# Autodesk Inventor assembly: rig
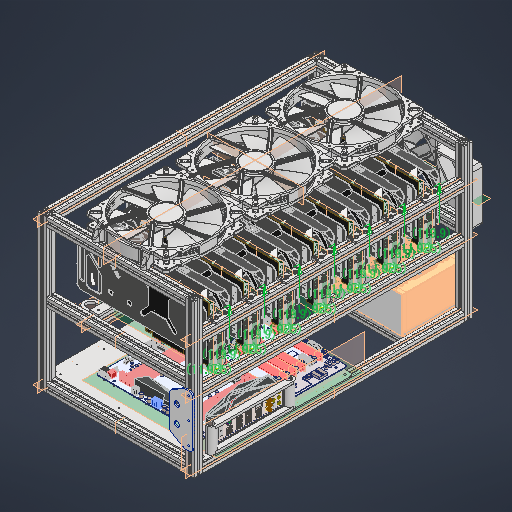
[picture p0: Inventor's stored thumbnail of the model, 512x512]
Saved by Autodesk Inventor 2026.2 (Build 302298010, 298A)
## iProperties
Created: 2026-05-30
Part Number: rig
Document SubType Name: Assembly
Designer: nyxeon
Author: nyxeon
## Documents named in this file (16)
- C:\Users\nyxeon\Documents\CAD\Inventor\eatx_case\robocup\rig.iam
- C:\Users\nyxeon\Documents\CAD\Inventor\eatx_case\robocup\l600.ipt
- C:\Users\nyxeon\Documents\CAD\Inventor\eatx_case\robocup\l320.ipt
- C:\Users\nyxeon\Documents\CAD\Inventor\eatx_case\robocup\l350.ipt
- C:\Users\nyxeon\Documents\CAD\Inventor\eatx_case\robocup\fan_unit_02.iam
- C:\Users\nyxeon\Documents\CAD\Inventor\eatx_case\robocup\fan_unit_01.iam
- C:\Users\nyxeon\Documents\CAD\Inventor\eatx_case\robocup\layout.iam
- C:\Users\nyxeon\Documents\CAD\Inventor\eatx_case\robocup\power_sync_module_case.ipt
- C:\Users\nyxeon\Documents\CAD\Inventor\eatx_case\robocup\power_sync_module_case_02.ipt
- C:\Users\nyxeon\Documents\CAD\Inventor\eatx_case\robocup\gpu_hold_plate.ipt
- C:\Users\nyxeon\Documents\CAD\Inventor\eatx_case\robocup\gpu_cable_holder.ipt
- C:\Users\nyxeon\Documents\CAD\Inventor\eatx_case\eatx_slim\resources\gpu\ASUS TUF RTX 3070 ti.iam
- C:\Users\nyxeon\Documents\CAD\Inventor\eatx_case\eatx_slim\resources\powersupply\ATX Power Supply v1.0.iam
- C:\Users\nyxeon\Documents\CAD\Inventor\eatx_case\robocup\gpu_support.ipt
- C:\Users\nyxeon\Documents\CAD\Inventor\eatx_case\robocup\atx_power_holder.ipt
- C:\Users\nyxeon\Documents\CAD\Inventor\eatx_case\robocup\robocup_power_sw_plate.ipt
## Components (49 placed, 15 different names)
1. l600:1 — フラッシュ:1, メイト:1, フラッシュ:2, メイト:2, フラッシュ:3, フラッシュ:4, メイト:43, フラッシュ:40
2. l600:2 — メイト:7, フラッシュ:13, フラッシュ:14, フラッシュ:28
3. l600:3 — メイト:3, フラッシュ:5, フラッシュ:6, メイト:4, フラッシュ:7, フラッシュ:8, メイト:8, メイト:20, フラッシュ:27, メイト:26, フラッシュ:30
4. l600:4 — メイト:8, メイト:9, フラッシュ:15, メイト:10
5. l600:5 — メイト:10, メイト:11, フラッシュ:16, メイト:28, フラッシュ:31, メイト:29, メイト:30, メイト:31, メイト:32, メイト:33, メイト:34, フラッシュ:32, フラッシュ:33, フラッシュ:34, フラッシュ:35, フラッシュ:36, フラッシュ:37
6. l320:1 — メイト:18, フラッシュ:23, フラッシュ:24, メイト:24
7. l320:2 — メイト:19, フラッシュ:25, フラッシュ:26, メイト:22, フラッシュ:29, メイト:25
8. l320:3 — メイト:20, フラッシュ:27, メイト:21
9. l320:4 — メイト:15, フラッシュ:20, フラッシュ:21, メイト:78
10. l320:5 — メイト:13, メイト:14, フラッシュ:19, フラッシュ:21, メイト:17, フラッシュ:22, フラッシュ:41, メイト:84
11. l320:6 — メイト:12, フラッシュ:17, フラッシュ:18, メイト:21, メイト:73, メイト:74, フラッシュ:55, メイト:79, メイト:80
12. l320:7 — メイト:5, メイト:6, フラッシュ:9, フラッシュ:10, フラッシュ:11, フラッシュ:12, メイト:13
13. l350:1 — フラッシュ:1, メイト:1, フラッシュ:2, メイト:5, フラッシュ:10, フラッシュ:11, メイト:7, フラッシュ:13, フラッシュ:14, メイト:14, フラッシュ:19, メイト:16, メイト:18, フラッシュ:23, フラッシュ:24
14. l350:2 — メイト:2, フラッシュ:3, フラッシュ:4, メイト:12, フラッシュ:17, フラッシュ:18, メイト:15, フラッシュ:20, メイト:19, フラッシュ:25, フラッシュ:26, メイト:23, メイト:76
15. l350:3 — メイト:3, フラッシュ:5, フラッシュ:6, メイト:6, フラッシュ:9, フラッシュ:12, メイト:9, フラッシュ:15, メイト:11, フラッシュ:16, メイト:27, メイト:35, メイト:83, フラッシュ:58
16. l350:4 — メイト:4, フラッシュ:7, フラッシュ:8, フラッシュ:54, メイト:75
17. l600:6 — メイト:16, メイト:17, フラッシュ:22, メイト:45, メイト:46, メイト:47, メイト:48, メイト:49, メイト:50, メイト:51, メイト:52, メイト:53, メイト:54, メイト:55, メイト:56, メイト:57, メイト:58, メイト:77, フラッシュ:56
18. fan_unit_02:1 [sub-assembly] — メイト:23, フラッシュ:29, メイト:25
19. fan_unit_01:1 [sub-assembly] — メイト:22, メイト:24, フラッシュ:28
20. layout:1 [sub-assembly] — メイト:26, メイト:27, フラッシュ:30, メイト:44
21. power_sync_module_case:1 — メイト:42, フラッシュ:38, フラッシュ:39, メイト:43, メイト:44, フラッシュ:40
22. power_sync_module_case_02:1 — メイト:42, フラッシュ:38, フラッシュ:39
23. gpu_hold_plate:1 — メイト:28, フラッシュ:31, メイト:35, メイト:36, メイト:59, メイト:60, 角度:1
24. gpu_hold_plate:2 — メイト:29, フラッシュ:32, メイト:36, メイト:37, メイト:61, メイト:62
25. gpu_hold_plate:3 — メイト:30, フラッシュ:33, メイト:37, メイト:38, メイト:63, メイト:64
26. gpu_hold_plate:4 — メイト:31, フラッシュ:34, メイト:38, メイト:39, メイト:65, メイト:66
27. gpu_hold_plate:5 — メイト:32, フラッシュ:35, メイト:39, メイト:40, メイト:69, メイト:70
28. gpu_hold_plate:6 — メイト:33, フラッシュ:36, メイト:40, メイト:41, メイト:67, メイト:68
29. gpu_hold_plate:7 — メイト:34, フラッシュ:37, メイト:41, メイト:71, メイト:72
30. gpu_cable_holder:1 — メイト:45, メイト:52, フラッシュ:41, フラッシュ:42
31. gpu_cable_holder:2 — メイト:46, メイト:53, フラッシュ:42, フラッシュ:43
32. gpu_cable_holder:3 — メイト:47, メイト:54, フラッシュ:43, フラッシュ:44
33. gpu_cable_holder:4 — メイト:48, メイト:55, フラッシュ:44, フラッシュ:45
34. gpu_cable_holder:5 — メイト:49, メイト:56, フラッシュ:45, フラッシュ:46
35. gpu_cable_holder:6 — メイト:50, メイト:57, フラッシュ:46, フラッシュ:47
36. gpu_cable_holder:7 — メイト:51, メイト:58, フラッシュ:47
37. ASUS TUF RTX 3070 ti:1 [sub-assembly] — メイト:71, メイト:72, フラッシュ:53
38. ASUS TUF RTX 3070 ti:2 [sub-assembly] — メイト:69, メイト:70, フラッシュ:52
39. ASUS TUF RTX 3070 ti:3 [sub-assembly] — メイト:67, メイト:68, フラッシュ:51, フラッシュ:53
40. ASUS TUF RTX 3070 ti:4 [sub-assembly] — メイト:65, メイト:66, フラッシュ:50, フラッシュ:51, フラッシュ:52
41. ASUS TUF RTX 3070 ti:5 [sub-assembly] — メイト:63, メイト:64, フラッシュ:49, フラッシュ:50
42. ASUS TUF RTX 3070 ti:6 [sub-assembly] — メイト:61, フラッシュ:48, メイト:62, フラッシュ:49
43. ASUS TUF RTX 3070 ti:7 [sub-assembly] — メイト:59, メイト:60, 角度:1, フラッシュ:48
44. ATX Power Supply v1.0:1 [sub-assembly] — メイト:74, フラッシュ:55, メイト:76, メイト:81
45. ATX Power Supply v1.0:2 [sub-assembly] — メイト:73, フラッシュ:54, メイト:75, メイト:82
46. gpu_support:1 — メイト:77, フラッシュ:56, メイト:78
47. atx_power_holder:1 — メイト:79, メイト:81, フラッシュ:57
48. atx_power_holder:2 — メイト:80, メイト:82, フラッシュ:57
49. robocup_power_sw_plate:1 — メイト:83, フラッシュ:58, メイト:84
## Relationships (143: Mate 84, Flush 58, Angle 1)
- フラッシュ:1 [Flush]: l600:1 ↔ l350:1
- メイト:1 [Mate]: l600:1 ↔ l350:1
- フラッシュ:2 [Flush]: l600:1 ↔ l350:1
- メイト:2 [Mate]: l600:1 ↔ l350:2
- フラッシュ:3 [Flush]: l600:1 ↔ l350:2
- フラッシュ:4 [Flush]: l600:1 ↔ l350:2
- メイト:3 [Mate]: l600:3 ↔ l350:3
- フラッシュ:5 [Flush]: l600:3 ↔ l350:3
- フラッシュ:6 [Flush]: l600:3 ↔ l350:3
- メイト:4 [Mate]: l600:3 ↔ l350:4
- フラッシュ:7 [Flush]: l600:3 ↔ l350:4
- フラッシュ:8 [Flush]: l600:3 ↔ l350:4
- メイト:5 [Mate]: l320:7 ↔ l350:1
- メイト:6 [Mate]: l320:7 ↔ l350:3
- フラッシュ:9 [Flush]: l320:7 ↔ l350:3
- フラッシュ:10 [Flush]: l320:7 ↔ l350:1
- フラッシュ:11 [Flush]: l320:7 ↔ l350:1
- フラッシュ:12 [Flush]: l320:7 ↔ l350:3
- メイト:7 [Mate]: l600:2 ↔ l350:1
- フラッシュ:13 [Flush]: l600:2 ↔ l350:1
- フラッシュ:14 [Flush]: l600:2 ↔ l350:1
- メイト:8 [Mate] (130 mm): l600:3 ↔ l600:4
- メイト:9 [Mate]: l600:4 ↔ l350:3
- フラッシュ:15 [Flush]: l600:4 ↔ l350:3
- メイト:10 [Mate] (90 mm): l600:4 ↔ l600:5
- メイト:11 [Mate]: l600:5 ↔ l350:3
- フラッシュ:16 [Flush]: l600:5 ↔ l350:3
- メイト:12 [Mate]: l320:6 ↔ l350:2
- フラッシュ:17 [Flush]: l320:6 ↔ l350:2
- フラッシュ:18 [Flush]: l320:6 ↔ l350:2
- メイト:13 [Mate] (150 mm): l320:5 ↔ l320:7
- メイト:14 [Mate]: l320:5 ↔ l350:1
- フラッシュ:19 [Flush]: l320:5 ↔ l350:1
- メイト:15 [Mate]: l320:4 ↔ l350:2
- フラッシュ:20 [Flush]: l320:4 ↔ l350:2
- フラッシュ:21 [Flush]: l320:4 ↔ l320:5
- メイト:16 [Mate] (80 mm): l350:1 ↔ l600:6
- メイト:17 [Mate]: l320:5 ↔ l600:6
- フラッシュ:22 [Flush]: l320:5 ↔ l600:6
- メイト:18 [Mate]: l320:1 ↔ l350:1
- フラッシュ:23 [Flush]: l320:1 ↔ l350:1
- フラッシュ:24 [Flush]: l320:1 ↔ l350:1
- メイト:19 [Mate]: l320:2 ↔ l350:2
- フラッシュ:25 [Flush]: l320:2 ↔ l350:2
- フラッシュ:26 [Flush]: l320:2 ↔ l350:2
- メイト:20 [Mate]: l600:3 ↔ l320:3
- フラッシュ:27 [Flush]: l600:3 ↔ l320:3
- メイト:21 [Mate] (100 mm): l320:3 ↔ l320:6
- メイト:22 [Mate]: l320:2 ↔ fan_unit_01:1
- メイト:23 [Mate]: l350:2 ↔ fan_unit_02:1
- メイト:24 [Mate]: l320:1 ↔ fan_unit_01:1
- フラッシュ:28 [Flush]: l600:2 ↔ fan_unit_01:1
- フラッシュ:29 [Flush]: l320:2 ↔ fan_unit_02:1
- メイト:25 [Mate]: l320:2 ↔ fan_unit_02:1
- メイト:26 [Mate]: l600:3 ↔ layout:1
- メイト:27 [Mate]: l350:3 ↔ layout:1
- フラッシュ:30 [Flush]: l600:3 ↔ layout:1
- メイト:28 [Mate]: l600:5 ↔ gpu_hold_plate:1
- フラッシュ:31 [Flush]: l600:5 ↔ gpu_hold_plate:1
- メイト:29 [Mate]: l600:5 ↔ gpu_hold_plate:2
- メイト:30 [Mate]: l600:5 ↔ gpu_hold_plate:3
- メイト:31 [Mate]: l600:5 ↔ gpu_hold_plate:4
- メイト:32 [Mate]: l600:5 ↔ gpu_hold_plate:5
- メイト:33 [Mate]: l600:5 ↔ gpu_hold_plate:6
- メイト:34 [Mate]: l600:5 ↔ gpu_hold_plate:7
- フラッシュ:32 [Flush]: l600:5 ↔ gpu_hold_plate:2
- フラッシュ:33 [Flush]: l600:5 ↔ gpu_hold_plate:3
- フラッシュ:34 [Flush]: l600:5 ↔ gpu_hold_plate:4
- フラッシュ:35 [Flush]: l600:5 ↔ gpu_hold_plate:5
- フラッシュ:36 [Flush]: l600:5 ↔ gpu_hold_plate:6
- フラッシュ:37 [Flush]: l600:5 ↔ gpu_hold_plate:7
- メイト:35 [Mate] (30 mm): l350:3 ↔ gpu_hold_plate:1
- メイト:36 [Mate] (40 mm): gpu_hold_plate:1 ↔ gpu_hold_plate:2
- メイト:37 [Mate] (40 mm): gpu_hold_plate:2 ↔ gpu_hold_plate:3
- メイト:38 [Mate] (40 mm): gpu_hold_plate:3 ↔ gpu_hold_plate:4
- メイト:39 [Mate] (40 mm): gpu_hold_plate:4 ↔ gpu_hold_plate:5
- メイト:40 [Mate] (40 mm): gpu_hold_plate:5 ↔ gpu_hold_plate:6
- メイト:41 [Mate] (40 mm): gpu_hold_plate:6 ↔ gpu_hold_plate:7
- メイト:42 [Mate]: power_sync_module_case:1 ↔ power_sync_module_case_02:1
- フラッシュ:38 [Flush]: power_sync_module_case:1 ↔ power_sync_module_case_02:1
- フラッシュ:39 [Flush]: power_sync_module_case:1 ↔ power_sync_module_case_02:1
- メイト:43 [Mate]: l600:1 ↔ power_sync_module_case:1
- メイト:44 [Mate]: layout:1 ↔ power_sync_module_case:1
- フラッシュ:40 [Flush] (-4.15 mm): l600:1 ↔ power_sync_module_case:1
- メイト:45 [Mate]: l600:6 ↔ gpu_cable_holder:1
- メイト:46 [Mate]: l600:6 ↔ gpu_cable_holder:2
- メイト:47 [Mate]: l600:6 ↔ gpu_cable_holder:3
- メイト:48 [Mate]: l600:6 ↔ gpu_cable_holder:4
- メイト:49 [Mate]: l600:6 ↔ gpu_cable_holder:5
- メイト:50 [Mate]: l600:6 ↔ gpu_cable_holder:6
- メイト:51 [Mate]: l600:6 ↔ gpu_cable_holder:7
- メイト:52 [Mate]: l600:6 ↔ gpu_cable_holder:1
- メイト:53 [Mate]: l600:6 ↔ gpu_cable_holder:2
- メイト:54 [Mate]: l600:6 ↔ gpu_cable_holder:3
- メイト:55 [Mate]: l600:6 ↔ gpu_cable_holder:4
- メイト:56 [Mate]: l600:6 ↔ gpu_cable_holder:5
- メイト:57 [Mate]: l600:6 ↔ gpu_cable_holder:6
- メイト:58 [Mate]: l600:6 ↔ gpu_cable_holder:7
- フラッシュ:41 [Flush] (-20 mm): l320:5 ↔ gpu_cable_holder:1
- フラッシュ:42 [Flush] (80.3 mm): gpu_cable_holder:1 ↔ gpu_cable_holder:2
- フラッシュ:43 [Flush] (80.3 mm): gpu_cable_holder:2 ↔ gpu_cable_holder:3
- フラッシュ:44 [Flush] (80.3 mm): gpu_cable_holder:3 ↔ gpu_cable_holder:4
- フラッシュ:45 [Flush] (80.3 mm): gpu_cable_holder:4 ↔ gpu_cable_holder:5
- フラッシュ:46 [Flush] (80.3 mm): gpu_cable_holder:5 ↔ gpu_cable_holder:6
- フラッシュ:47 [Flush] (80.3 mm): gpu_cable_holder:6 ↔ gpu_cable_holder:7
- メイト:59 [Mate]: gpu_hold_plate:1 ↔ ASUS TUF RTX 3070 ti:7
- メイト:60 [Mate]: gpu_hold_plate:1 ↔ ASUS TUF RTX 3070 ti:7
- 角度:1 [Angle] (0 deg): gpu_hold_plate:1 ↔ ASUS TUF RTX 3070 ti:7
- メイト:61 [Mate]: gpu_hold_plate:2 ↔ ASUS TUF RTX 3070 ti:6
- フラッシュ:48 [Flush]: ASUS TUF RTX 3070 ti:6 ↔ ASUS TUF RTX 3070 ti:7
- メイト:62 [Mate]: gpu_hold_plate:2 ↔ ASUS TUF RTX 3070 ti:6
- メイト:63 [Mate]: gpu_hold_plate:3 ↔ ASUS TUF RTX 3070 ti:5
- メイト:64 [Mate]: gpu_hold_plate:3 ↔ ASUS TUF RTX 3070 ti:5
- フラッシュ:49 [Flush]: ASUS TUF RTX 3070 ti:5 ↔ ASUS TUF RTX 3070 ti:6
- メイト:65 [Mate]: gpu_hold_plate:4 ↔ ASUS TUF RTX 3070 ti:4
- メイト:66 [Mate]: gpu_hold_plate:4 ↔ ASUS TUF RTX 3070 ti:4
- フラッシュ:50 [Flush]: ASUS TUF RTX 3070 ti:4 ↔ ASUS TUF RTX 3070 ti:5
- メイト:67 [Mate]: gpu_hold_plate:6 ↔ ASUS TUF RTX 3070 ti:3
- メイト:68 [Mate]: gpu_hold_plate:6 ↔ ASUS TUF RTX 3070 ti:3
- フラッシュ:51 [Flush]: ASUS TUF RTX 3070 ti:3 ↔ ASUS TUF RTX 3070 ti:4
- メイト:69 [Mate]: gpu_hold_plate:5 ↔ ASUS TUF RTX 3070 ti:2
- メイト:70 [Mate]: gpu_hold_plate:5 ↔ ASUS TUF RTX 3070 ti:2
- フラッシュ:52 [Flush]: ASUS TUF RTX 3070 ti:2 ↔ ASUS TUF RTX 3070 ti:4
- メイト:71 [Mate]: gpu_hold_plate:7 ↔ ASUS TUF RTX 3070 ti:1
- メイト:72 [Mate]: gpu_hold_plate:7 ↔ ASUS TUF RTX 3070 ti:1
- フラッシュ:53 [Flush]: ASUS TUF RTX 3070 ti:1 ↔ ASUS TUF RTX 3070 ti:3
- メイト:73 [Mate]: l320:6 ↔ ATX Power Supply v1.0:2
- メイト:74 [Mate]: l320:6 ↔ ATX Power Supply v1.0:1
- フラッシュ:54 [Flush]: l350:4 ↔ ATX Power Supply v1.0:2
- フラッシュ:55 [Flush]: l320:6 ↔ ATX Power Supply v1.0:1
- メイト:75 [Mate]: l350:4 ↔ ATX Power Supply v1.0:2
- メイト:76 [Mate]: l350:2 ↔ ATX Power Supply v1.0:1
- メイト:77 [Mate]: l600:6 ↔ gpu_support:1
- フラッシュ:56 [Flush]: l600:6 ↔ gpu_support:1
- メイト:78 [Mate]: l320:4 ↔ gpu_support:1
- メイト:79 [Mate]: l320:6 ↔ atx_power_holder:1
- メイト:80 [Mate]: l320:6 ↔ atx_power_holder:2
- メイト:81 [Mate]: ATX Power Supply v1.0:1 ↔ atx_power_holder:1
- メイト:82 [Mate]: ATX Power Supply v1.0:2 ↔ atx_power_holder:2
- フラッシュ:57 [Flush]: atx_power_holder:1 ↔ atx_power_holder:2
- メイト:83 [Mate]: l350:3 ↔ robocup_power_sw_plate:1
- フラッシュ:58 [Flush]: l350:3 ↔ robocup_power_sw_plate:1
- メイト:84 [Mate]: l320:5 ↔ robocup_power_sw_plate:1
